# Autodesk Inventor assembly: 2AM-17-A-6200 - claw arm
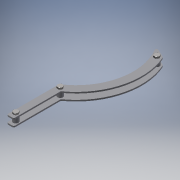
[picture p0: Inventor's stored thumbnail of the model, 180x180]
Saved by Autodesk Inventor 2017 (Build 210142000, 142)
## iProperties
Created: 2017-12-27
Part Number: 2AM-17-A-6200 - claw arm
Document SubType Name: Assembly
Designer: Micah
Author: Micah
## Documents named in this file (4)
- C:\Users\Micah\Desktop\inventor\CADathon-2017\2AM-17-A-0200 - Smokestack Elevator\2AM-17-A-6200 - claw arm.iam
- C:\Users\Micah\Desktop\inventor\CADathon-2017\2AM-17-A-0200 - Smokestack Elevator\2AM-17-P-5201 - claw arm.ipt
- C:\Users\Micah\Desktop\inventor\CADathon-2017\2AM-17-A-0200 - Smokestack Elevator\2AM-17-P-5202 - arm supports.ipt
- C:\Users\Micah\Documents\Inventor\Content Center Files\R2017\en-US\AS 2465(2)\AS 2465 - 1_4 x 1_2  UNC.ipt
## Components (8 placed, 3 different names)
1. 2AM-17-P-5201 - claw arm:1 — Mate:4, Insert:1, Insert:2, Insert:3
2. 2AM-17-P-5201 - claw arm:2 — Mate:1, Mate:2, Mate:3
3. 2AM-17-P-5202 - arm supports:1 — Mate:1, Mate:4
4. 2AM-17-P-5202 - arm supports:2 — Mate:2
5. 2AM-17-P-5202 - arm supports:3 — Mate:3
6. AS 2465 - Inch 1/4 x 1/2  UNC:1 — Insert:1
7. AS 2465 - Inch 1/4 x 1/2  UNC:2 — Insert:2
8. AS 2465 - Inch 1/4 x 1/2  UNC:3 — Insert:3
## Relationships (7: Mate 4, Insert 3)
- Mate:1: 2AM-17-P-5201 - claw arm:2 ↔ 2AM-17-P-5202 - arm supports:1
- Mate:2: 2AM-17-P-5201 - claw arm:2 ↔ 2AM-17-P-5202 - arm supports:2
- Mate:3: 2AM-17-P-5201 - claw arm:2 ↔ 2AM-17-P-5202 - arm supports:3
- Mate:4: 2AM-17-P-5201 - claw arm:1 ↔ 2AM-17-P-5202 - arm supports:1
- Insert:1: 2AM-17-P-5201 - claw arm:1 ↔ AS 2465 - Inch 1/4 x 1/2  UNC:1
- Insert:2: 2AM-17-P-5201 - claw arm:1 ↔ AS 2465 - Inch 1/4 x 1/2  UNC:2
- Insert:3: 2AM-17-P-5201 - claw arm:1 ↔ AS 2465 - Inch 1/4 x 1/2  UNC:3
